# Autodesk Inventor assembly: Parametric
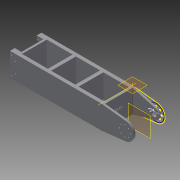
[picture p0: Inventor's stored thumbnail of the model, 180x180]
Saved by Autodesk Inventor 2015 (Build 190159000, 159)
## iProperties
Created: 2017-01-04
Part Number: Parametric
Document SubType Name: Assembly
Designer: Rudge-Top
Author: Rudge-Top
## Documents named in this file (4)
- C:\Users\Rudge-Top\Documents\RoboticArm\Inventor 2015\Straight Links\Parametric.iam
- C:\Users\Rudge-Top\Documents\RoboticArm\Inventor 2015\Straight Links\Parametric.ipt
- C:\Users\Rudge-Top\Documents\RoboticArm\Inventor 2015\Mounts\BaseMount.ipt
- C:\Users\Rudge-Top\Documents\RoboticArm\Inventor 2015\Mounts\Turnmount.ipt
## Components (3 placed, 3 different names)
1. Parametric:1 — Mate:1, Flush:1, Flush:2, Mate:2, Flush:3, Flush:4
2. BaseMount:1 — Mate:2, Flush:3, Flush:4
3. Turnmount:1 — Mate:1, Flush:1, Flush:2
## Relationships (6: Flush 4, Mate 2)
- Mate:1: Parametric:1 ↔ Turnmount:1
- Flush:1: Parametric:1 ↔ Turnmount:1
- Flush:2: Parametric:1 ↔ Turnmount:1
- Mate:2: Parametric:1 ↔ BaseMount:1
- Flush:3: Parametric:1 ↔ BaseMount:1
- Flush:4: Parametric:1 ↔ BaseMount:1
